# Autodesk Inventor assembly: Assembly12
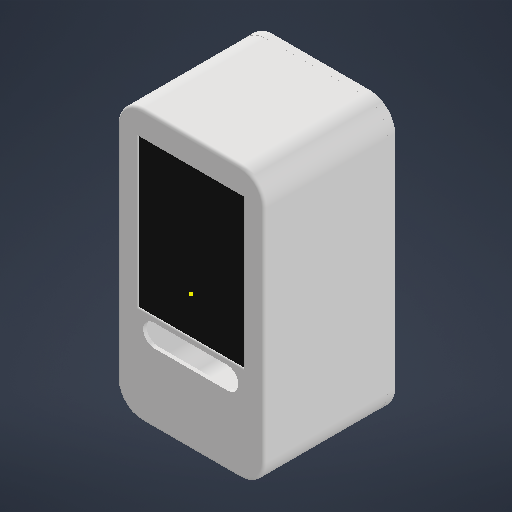
[picture p0: Inventor's stored thumbnail of the model, 512x512]
Saved by Autodesk Inventor 2026 (Build 300175050, 175E)
## iProperties
Created: 2026-03-28
Part Number: Assembly12
Document SubType Name: Assembly
Designer: tp2105
Author: tp2105
## Documents named in this file (4)
- C:\Users\tp2105\OneDrive - University of Bath\Hackathon\Assembly12.iam
- C:\Users\tp2105\OneDrive - University of Bath\Hackathon\MainBody.ipt
- C:\Users\tp2105\OneDrive - University of Bath\Hackathon\BackPlate.ipt
- C:\Users\tp2105\OneDrive - University of Bath\Hackathon\OLED.ipt
## Components (3 placed, 3 different names)
1. MainBody:1 — Mate:1, Mate:2, Mate:3, Mate:4
2. BackPlate:1 — Mate:1, Mate:2
3. OLED:1 — Mate:3, Mate:4
## Relationships (4: Mate 4)
- Mate:1: MainBody:1 ↔ BackPlate:1
- Mate:2: MainBody:1 ↔ BackPlate:1
- Mate:3: MainBody:1 ↔ OLED:1
- Mate:4: MainBody:1 ↔ OLED:1
